# Autodesk Inventor assembly: teststructure1
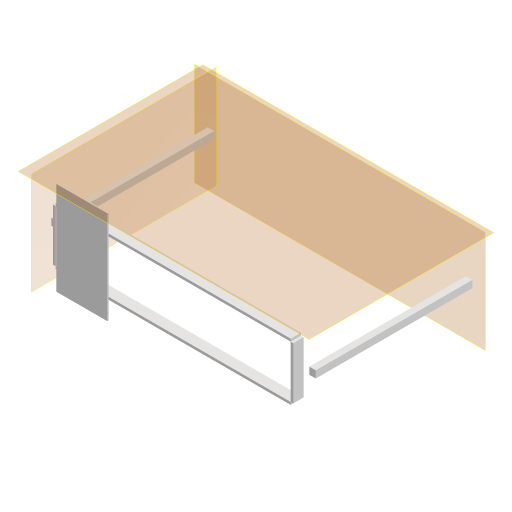
[picture p0: Inventor's stored thumbnail of the model, 512x512]
Saved by Autodesk Inventor 2024 (Build 280153000, 153)
## iProperties
Created: 2024-02-23
Part Number: teststructure1
Document SubType Name: Assembly
Designer: Frank
Author: Frank
## Documents named in this file (5)
- C:\Users\Cex\OneDrive\OneDrive - University of Bristol\Documents\Year_5\DP5\Agrivoltaicmodel\CAD\teststructure1.iam
- C:\Users\Cex\OneDrive\OneDrive - University of Bristol\Documents\Year_5\DP5\Agrivoltaicmodel\CAD\boxsectiontest.ipt
- C:\Users\Cex\OneDrive\OneDrive - University of Bristol\Documents\Year_5\DP5\Agrivoltaicmodel\CAD\testpanel.ipt
- C:\Users\Cex\OneDrive\OneDrive - University of Bristol\Documents\Year_5\DP5\Agrivoltaicmodel\CAD\boxsectiontestcross.ipt
- C:\Users\Cex\OneDrive\OneDrive - University of Bristol\Documents\Year_5\DP5\Agrivoltaicmodel\CAD\pylon.ipt
## Components (7 placed, 4 different names)
1. boxsectiontest:1 — Mate:4, Flush:2, Mate:10, Flush:3, Mate:13, Mate:14, Mate:20
2. boxsectiontest:2 — Flush:1, Mate:9, Mate:11, Mate:12, Mate:15, Mate:18
3. testpanel:2 — Mate:18, Mate:20, Flush:5
4. boxsectiontestcross:1 — Mate:9, Mate:10, Flush:3, Mate:11, Mate:14, Mate:15, Mate:16, Mate:23
5. boxsectiontestcross:2 — Flush:1, Mate:4, Flush:2, Mate:8, Mate:12, Mate:13, Mate:22, Flush:6
6. pylon:1 — Mate:5, Mate:16, Flush:4, Mate:23
7. pylon:2 — Mate:6, Mate:8, Flush:4, Mate:21, Mate:22, Flush:6
## Relationships (23: Mate 17, Flush 6)
- Flush:1: boxsectiontest:2 ↔ boxsectiontestcross:2
- Mate:4 (2.5 mm): boxsectiontest:1 ↔ boxsectiontestcross:2
- Mate:5: pylon:1
- Mate:6: pylon:2
- Flush:2: boxsectiontest:1 ↔ boxsectiontestcross:2
- Mate:8: boxsectiontestcross:2 ↔ pylon:2
- Mate:9: boxsectiontest:2 ↔ boxsectiontestcross:1
- Mate:10: boxsectiontest:1 ↔ boxsectiontestcross:1
- Flush:3: boxsectiontest:1 ↔ boxsectiontestcross:1
- Mate:11 (2.5 mm): boxsectiontest:2 ↔ boxsectiontestcross:1
- Mate:12 (2.5 mm): boxsectiontest:2 ↔ boxsectiontestcross:2
- Mate:13 (2.5 mm): boxsectiontest:1 ↔ boxsectiontestcross:2
- Mate:14 (2.5 mm): boxsectiontest:1 ↔ boxsectiontestcross:1
- Mate:15 (2.5 mm): boxsectiontest:2 ↔ boxsectiontestcross:1
- Mate:16: boxsectiontestcross:1 ↔ pylon:1
- Flush:4: pylon:1 ↔ pylon:2
- Mate:18: boxsectiontest:2 ↔ testpanel:2
- Mate:20 (463.5 mm): boxsectiontest:1 ↔ testpanel:2
- Mate:21: pylon:2
- Flush:5: testpanel:2
- Mate:22 (146.8 mm): boxsectiontestcross:2 ↔ pylon:2
- Mate:23 (146.8 mm): boxsectiontestcross:1 ↔ pylon:1
- Flush:6 (574.75 mm): boxsectiontestcross:2 ↔ pylon:2
